# Autodesk Inventor assembly: mesoSPIM_excitation_path_optics_V1
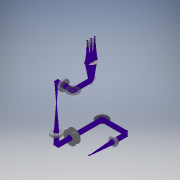
[picture p0: Inventor's stored thumbnail of the model, 180x180]
Saved by Autodesk Inventor 2016 (Build 200138000, 138)
## iProperties
Company: Unknown
Created: 2018-08-27
Part Number: mesoSPIM_excitation_path_optics_V1
Document SubType Name: Assembly
Designer: voigt
Sending System: HarmonyWare Translators
Preprocessor: HarmonyWare STEP v1.9.13
Title: D:\Microscope_Design\CAD_Files\mesoSPIM_design\mesoSPIM\optical_design\mesoSPIM_excitation_path_optics_V1.STP
Author: Unknown
## Documents named in this file (71)
- D:\Microscope_Design\CAD_Files\mesoSPIM_design\mesoSPIM\optical_design\cad_export_v1\mesoSPIM_excitation_path_optics_V1.iam
- D:\Microscope_Design\CAD_Files\mesoSPIM_design\mesoSPIM\optical_design\cad_export_v1\NONE.ipt
- D:\Microscope_Design\CAD_Files\mesoSPIM_design\mesoSPIM\optical_design\cad_export_v1\NONE_1.ipt
- D:\Microscope_Design\CAD_Files\mesoSPIM_design\mesoSPIM\optical_design\cad_export_v1\NONE_2.ipt
- D:\Microscope_Design\CAD_Files\mesoSPIM_design\mesoSPIM\optical_design\cad_export_v1\NONE_3.ipt
- D:\Microscope_Design\CAD_Files\mesoSPIM_design\mesoSPIM\optical_design\cad_export_v1\NONE_4.ipt
- D:\Microscope_Design\CAD_Files\mesoSPIM_design\mesoSPIM\optical_design\cad_export_v1\NONE_5.ipt
- D:\Microscope_Design\CAD_Files\mesoSPIM_design\mesoSPIM\optical_design\cad_export_v1\NONE_6.ipt
- D:\Microscope_Design\CAD_Files\mesoSPIM_design\mesoSPIM\optical_design\cad_export_v1\NONE_7.ipt
- D:\Microscope_Design\CAD_Files\mesoSPIM_design\mesoSPIM\optical_design\cad_export_v1\NONE_8.ipt
- D:\Microscope_Design\CAD_Files\mesoSPIM_design\mesoSPIM\optical_design\cad_export_v1\NONE_9.ipt
- D:\Microscope_Design\CAD_Files\mesoSPIM_design\mesoSPIM\optical_design\cad_export_v1\NONE_10.ipt
- D:\Microscope_Design\CAD_Files\mesoSPIM_design\mesoSPIM\optical_design\cad_export_v1\NONE_11.ipt
- D:\Microscope_Design\CAD_Files\mesoSPIM_design\mesoSPIM\optical_design\cad_export_v1\NONE_12.ipt
- D:\Microscope_Design\CAD_Files\mesoSPIM_design\mesoSPIM\optical_design\cad_export_v1\NONE_13.ipt
- D:\Microscope_Design\CAD_Files\mesoSPIM_design\mesoSPIM\optical_design\cad_export_v1\NONE_14.ipt
- D:\Microscope_Design\CAD_Files\mesoSPIM_design\mesoSPIM\optical_design\cad_export_v1\NONE_15.ipt
- D:\Microscope_Design\CAD_Files\mesoSPIM_design\mesoSPIM\optical_design\cad_export_v1\NONE_16.ipt
- D:\Microscope_Design\CAD_Files\mesoSPIM_design\mesoSPIM\optical_design\cad_export_v1\NONE_17.ipt
- D:\Microscope_Design\CAD_Files\mesoSPIM_design\mesoSPIM\optical_design\cad_export_v1\NONE_18.ipt
- D:\Microscope_Design\CAD_Files\mesoSPIM_design\mesoSPIM\optical_design\cad_export_v1\NONE_19.ipt
- D:\Microscope_Design\CAD_Files\mesoSPIM_design\mesoSPIM\optical_design\cad_export_v1\NONE_20.ipt
- D:\Microscope_Design\CAD_Files\mesoSPIM_design\mesoSPIM\optical_design\cad_export_v1\NONE_21.ipt
- D:\Microscope_Design\CAD_Files\mesoSPIM_design\mesoSPIM\optical_design\cad_export_v1\NONE_22.ipt
- D:\Microscope_Design\CAD_Files\mesoSPIM_design\mesoSPIM\optical_design\cad_export_v1\NONE_23.ipt
- D:\Microscope_Design\CAD_Files\mesoSPIM_design\mesoSPIM\optical_design\cad_export_v1\NONE_24.ipt
- D:\Microscope_Design\CAD_Files\mesoSPIM_design\mesoSPIM\optical_design\cad_export_v1\NONE_25.ipt
- D:\Microscope_Design\CAD_Files\mesoSPIM_design\mesoSPIM\optical_design\cad_export_v1\NONE_26.ipt
- D:\Microscope_Design\CAD_Files\mesoSPIM_design\mesoSPIM\optical_design\cad_export_v1\NONE_27.ipt
- D:\Microscope_Design\CAD_Files\mesoSPIM_design\mesoSPIM\optical_design\cad_export_v1\NONE_28.ipt
- D:\Microscope_Design\CAD_Files\mesoSPIM_design\mesoSPIM\optical_design\cad_export_v1\NONE_29.ipt
- D:\Microscope_Design\CAD_Files\mesoSPIM_design\mesoSPIM\optical_design\cad_export_v1\NONE_30.ipt
- D:\Microscope_Design\CAD_Files\mesoSPIM_design\mesoSPIM\optical_design\cad_export_v1\NONE_31.ipt
- D:\Microscope_Design\CAD_Files\mesoSPIM_design\mesoSPIM\optical_design\cad_export_v1\NONE_32.ipt
- D:\Microscope_Design\CAD_Files\mesoSPIM_design\mesoSPIM\optical_design\cad_export_v1\NONE_33.ipt
- D:\Microscope_Design\CAD_Files\mesoSPIM_design\mesoSPIM\optical_design\cad_export_v1\NONE_34.ipt
- D:\Microscope_Design\CAD_Files\mesoSPIM_design\mesoSPIM\optical_design\cad_export_v1\NONE_35.ipt
- D:\Microscope_Design\CAD_Files\mesoSPIM_design\mesoSPIM\optical_design\cad_export_v1\NONE_36.ipt
- D:\Microscope_Design\CAD_Files\mesoSPIM_design\mesoSPIM\optical_design\cad_export_v1\NONE_37.ipt
- D:\Microscope_Design\CAD_Files\mesoSPIM_design\mesoSPIM\optical_design\cad_export_v1\NONE_38.ipt
- D:\Microscope_Design\CAD_Files\mesoSPIM_design\mesoSPIM\optical_design\cad_export_v1\NONE_39.ipt
- D:\Microscope_Design\CAD_Files\mesoSPIM_design\mesoSPIM\optical_design\cad_export_v1\NONE_40.ipt
- D:\Microscope_Design\CAD_Files\mesoSPIM_design\mesoSPIM\optical_design\cad_export_v1\NONE_41.ipt
- D:\Microscope_Design\CAD_Files\mesoSPIM_design\mesoSPIM\optical_design\cad_export_v1\NONE_42.ipt
- D:\Microscope_Design\CAD_Files\mesoSPIM_design\mesoSPIM\optical_design\cad_export_v1\NONE_43.ipt
- D:\Microscope_Design\CAD_Files\mesoSPIM_design\mesoSPIM\optical_design\cad_export_v1\NONE_44.ipt
- D:\Microscope_Design\CAD_Files\mesoSPIM_design\mesoSPIM\optical_design\cad_export_v1\NONE_45.ipt
- D:\Microscope_Design\CAD_Files\mesoSPIM_design\mesoSPIM\optical_design\cad_export_v1\NONE_46.ipt
- D:\Microscope_Design\CAD_Files\mesoSPIM_design\mesoSPIM\optical_design\cad_export_v1\NONE_47.ipt
- D:\Microscope_Design\CAD_Files\mesoSPIM_design\mesoSPIM\optical_design\cad_export_v1\NONE_48.ipt
- D:\Microscope_Design\CAD_Files\mesoSPIM_design\mesoSPIM\optical_design\cad_export_v1\NONE_49.ipt
- D:\Microscope_Design\CAD_Files\mesoSPIM_design\mesoSPIM\optical_design\cad_export_v1\NONE_50.ipt
- D:\Microscope_Design\CAD_Files\mesoSPIM_design\mesoSPIM\optical_design\cad_export_v1\NONE_51.ipt
- D:\Microscope_Design\CAD_Files\mesoSPIM_design\mesoSPIM\optical_design\cad_export_v1\NONE_52.ipt
- D:\Microscope_Design\CAD_Files\mesoSPIM_design\mesoSPIM\optical_design\cad_export_v1\NONE_53.ipt
- D:\Microscope_Design\CAD_Files\mesoSPIM_design\mesoSPIM\optical_design\cad_export_v1\NONE_54.ipt
- D:\Microscope_Design\CAD_Files\mesoSPIM_design\mesoSPIM\optical_design\cad_export_v1\NONE_55.ipt
- D:\Microscope_Design\CAD_Files\mesoSPIM_design\mesoSPIM\optical_design\cad_export_v1\NONE_56.ipt
- D:\Microscope_Design\CAD_Files\mesoSPIM_design\mesoSPIM\optical_design\cad_export_v1\NONE_57.ipt
- D:\Microscope_Design\CAD_Files\mesoSPIM_design\mesoSPIM\optical_design\cad_export_v1\NONE_58.ipt
- D:\Microscope_Design\CAD_Files\mesoSPIM_design\mesoSPIM\optical_design\cad_export_v1\NONE_59.ipt
- D:\Microscope_Design\CAD_Files\mesoSPIM_design\mesoSPIM\optical_design\cad_export_v1\NONE_60.ipt
- D:\Microscope_Design\CAD_Files\mesoSPIM_design\mesoSPIM\optical_design\cad_export_v1\NONE_61.ipt
- D:\Microscope_Design\CAD_Files\mesoSPIM_design\mesoSPIM\optical_design\cad_export_v1\NONE_62.ipt
- D:\Microscope_Design\CAD_Files\mesoSPIM_design\mesoSPIM\optical_design\cad_export_v1\NONE_63.ipt
- D:\Microscope_Design\CAD_Files\mesoSPIM_design\mesoSPIM\optical_design\cad_export_v1\NONE_64.ipt
- D:\Microscope_Design\CAD_Files\mesoSPIM_design\mesoSPIM\optical_design\cad_export_v1\NONE_65.ipt
- D:\Microscope_Design\CAD_Files\mesoSPIM_design\mesoSPIM\optical_design\cad_export_v1\NONE_66.ipt
- D:\Microscope_Design\CAD_Files\mesoSPIM_design\mesoSPIM\optical_design\cad_export_v1\NONE_67.ipt
- D:\Microscope_Design\CAD_Files\mesoSPIM_design\mesoSPIM\optical_design\cad_export_v1\NONE_68.ipt
- D:\Microscope_Design\CAD_Files\mesoSPIM_design\mesoSPIM\optical_design\cad_export_v1\NONE_69.ipt
## Components (70 placed, 70 different names)
1. NONE
2. NONE_1
3. NONE_2
4. NONE_3
5. NONE_4
6. NONE_5
7. NONE_6
8. NONE_7
9. NONE_8
10. NONE_9
11. NONE_10
12. NONE_11
13. NONE_12
14. NONE_13
15. NONE_14
16. NONE_15
17. NONE_16
18. NONE_17
19. NONE_18
20. NONE_19
21. NONE_20
22. NONE_21
23. NONE_22
24. NONE_23
25. NONE_24 — Mate:2
26. NONE_25
27. NONE_26
28. NONE_27
29. NONE_28
30. NONE_29
31. NONE_30
32. NONE_31
33. NONE_32
34. NONE_33
35. NONE_34
36. NONE_35
37. NONE_36
38. NONE_37
39. NONE_38
40. NONE_39
41. NONE_40
42. NONE_41
43. NONE_42
44. NONE_43
45. NONE_44
46. NONE_45
47. NONE_46
48. NONE_47
49. NONE_48
50. NONE_49
51. NONE_50
52. NONE_51
53. NONE_52
54. NONE_53 — Mate:1
55. NONE_54
56. NONE_55
57. NONE_56
58. NONE_57
59. NONE_58
60. NONE_59
61. NONE_60
62. NONE_61
63. NONE_62
64. NONE_63
65. NONE_64
66. NONE_65
67. NONE_66
68. NONE_67
69. NONE_68
70. NONE_69
## Relationships (2: Mate 2)
- Mate:1: NONE_53
- Mate:2: NONE_24
